# Autodesk Inventor assembly: Matchboxscope_v1
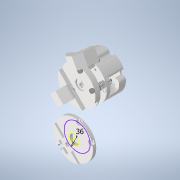
[picture p0: Inventor's stored thumbnail of the model, 180x180]
Saved by Autodesk Inventor 2022 (Build 260153000, 153)
## iProperties
Created: 2022-04-02
Part Number: Matchboxscope_v1
Document SubType Name: Assembly
Designer: Prakash Lab
Author: Prakash Lab
## Documents named in this file (11)
- C:\Users\diederichbenedict\Dropbox\Dokumente\Promotion\PROJECTS\Matchboxscope\INVENTOR\Matchboxscope_v1.iam
- C:\Users\diederichbenedict\Dropbox\Dokumente\Promotion\PROJECTS\Matchboxscope\INVENTOR\Matchboxscope_Lightperiscope_V0.ipt
- C:\Users\diederichbenedict\Dropbox\Dokumente\Promotion\PROJECTS\Matchboxscope\INVENTOR\Matchboxscope_Lightperiscope_long_V0.ipt
- C:\Users\diederichbenedict\Dropbox\Dokumente\Promotion\PROJECTS\Matchboxscope\INVENTOR\Matchboxscope_bottom_v0.ipt
- C:\Users\diederichbenedict\Dropbox\Dokumente\Promotion\PROJECTS\Matchboxscope\INVENTOR\00_ESP3-CAM.iam
- C:\Users\diederichbenedict\Dropbox\Dokumente\Promotion\PROJECTS\Matchboxscope\INVENTOR\Matchboxscope_sample_v1.ipt
- C:\Users\diederichbenedict\Dropbox\Dokumente\Promotion\PROJECTS\Matchboxscope\INVENTOR\00_Powerbank.ipt
- C:\Users\diederichbenedict\Dropbox\Dokumente\Promotion\PROJECTS\Matchboxscope\INVENTOR\00_spring.ipt
- C:\Users\diederichbenedict\Documents\Inventor\Content Center Files\R2022\de-DE\DIN 912\DIN 912 - M3 x 0.5 x 25 x 18.ipt
- C:\Users\diederichbenedict\Dropbox\Dokumente\Promotion\PROJECTS\Matchboxscope\INVENTOR\Matchboxscope_middle2_v2.ipt
- C:\Users\diederichbenedict\Dropbox\Dokumente\Promotion\PROJECTS\Matchboxscope\INVENTOR\Matchboxscope_sample_universal.ipt
## Components (18 placed, 10 different names)
1. Matchboxscope_Lightperiscope_V0:1
2. Matchboxscope_Lightperiscope_long_V0:1 — Angle:2, Einfügen:10, Fluchtend:2
3. Matchboxscope_bottom_v0:1 — Mate:1, Mate:2, Mate:3, Mate:4, Flush:1, Einfügen:11, Passend:7, Winkel:3
4. 00_ESP3-CAM:1 [sub-assembly] — Mate:4, Flush:1
5. Matchboxscope_sample_v1:1 — Angle:2, Einfügen:10, Passend:8, Winkel:3, Einfügen:12, Einfügen:13, Einfügen:14, Einfügen:15, Einfügen:16, Einfügen:17, Fluchtend:2
6. 00_Powerbank:1
7. 00_spring:1 — Einfügen:17
8. DIN 912 - ersetzt durch DIN EN ISO 4762 M3 x 25:1 — Einfügen:14
9. DIN 912 - ersetzt durch DIN EN ISO 4762 M3 x 25:2 — Einfügen:12
10. DIN 912 - ersetzt durch DIN EN ISO 4762 M3 x 25:3 — Einfügen:13
11. 00_spring:3 — Einfügen:15
12. 00_spring:4 — Einfügen:16
13. DIN 912 - ersetzt durch DIN EN ISO 4762 M3 x 25:4
14. DIN 912 - ersetzt durch DIN EN ISO 4762 M3 x 25:5
15. DIN 912 - ersetzt durch DIN EN ISO 4762 M3 x 25:6
16. DIN 912 - ersetzt durch DIN EN ISO 4762 M3 x 25:7
17. Matchboxscope_middle2_v2:1 — Einfügen:11, Passend:7, Passend:8
18. Matchboxscope_sample_universal:1
## Relationships (18: Insert 8, Mate 6, Flush 2, Angle 2)
- Mate:1: Matchboxscope_bottom_v0:1
- Mate:2: Matchboxscope_bottom_v0:1
- Mate:3: Matchboxscope_bottom_v0:1
- Mate:4: Matchboxscope_bottom_v0:1 ↔ 00_ESP3-CAM:1
- Flush:1: Matchboxscope_bottom_v0:1 ↔ 00_ESP3-CAM:1
- Angle:2 (90 deg): Matchboxscope_Lightperiscope_long_V0:1 ↔ Matchboxscope_sample_v1:1
- Einfügen:10 [Insert]: Matchboxscope_Lightperiscope_long_V0:1 ↔ Matchboxscope_sample_v1:1
- Einfügen:11 [Insert]: Matchboxscope_bottom_v0:1 ↔ Matchboxscope_middle2_v2:1
- Passend:7 [Mate]: Matchboxscope_bottom_v0:1 ↔ Matchboxscope_middle2_v2:1
- Passend:8 [Mate]: Matchboxscope_sample_v1:1 ↔ Matchboxscope_middle2_v2:1
- Winkel:3 [Angle] (45 deg): Matchboxscope_bottom_v0:1 ↔ Matchboxscope_sample_v1:1
- Einfügen:12 [Insert]: Matchboxscope_sample_v1:1 ↔ DIN 912 - ersetzt durch DIN EN ISO 4762 M3 x 25:2
- Einfügen:13 [Insert]: Matchboxscope_sample_v1:1 ↔ DIN 912 - ersetzt durch DIN EN ISO 4762 M3 x 25:3
- Einfügen:14 [Insert]: Matchboxscope_sample_v1:1 ↔ DIN 912 - ersetzt durch DIN EN ISO 4762 M3 x 25:1
- Einfügen:15 [Insert]: Matchboxscope_sample_v1:1 ↔ 00_spring:3
- Einfügen:16 [Insert]: Matchboxscope_sample_v1:1 ↔ 00_spring:4
- Einfügen:17 [Insert]: Matchboxscope_sample_v1:1 ↔ 00_spring:1
- Fluchtend:2 [Flush]: Matchboxscope_Lightperiscope_long_V0:1 ↔ Matchboxscope_sample_v1:1
